# Autodesk Inventor assembly: om_AssemblyBody
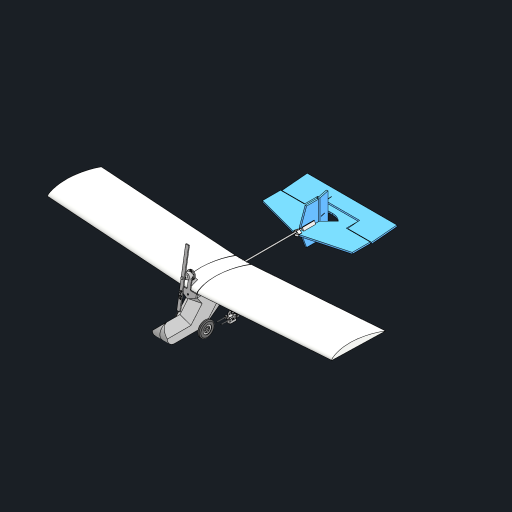
[picture p0: Inventor's stored thumbnail of the model, 512x512]
Saved by Autodesk Inventor 2023 (Build 270158000, 158)
## iProperties
Created: 2022-06-19
Part Number: om_AssemblyBody
Document SubType Name: Assembly
Designer: legot
Author: legot
## Documents named in this file (17)
- C:\Users\legot\OneDrive\ドキュメント\Inventor\HIKOSAPO\OM\om_HIKOROBO.iam
- C:\Users\legot\OneDrive\ドキュメント\Inventor\HIKOSAPO\OM\om_Body_L.ipt
- C:\Users\legot\OneDrive\ドキュメント\Inventor\HIKOSAPO\OM\om_Body_R.ipt
- C:\Users\legot\OneDrive\ドキュメント\Inventor\HIKOSAPO\OM\om_MotorMount.ipt
- C:\Users\legot\OneDrive\ドキュメント\Inventor\HIKOSAPO\public_parts\MainMotor.ipt
- C:\Users\legot\OneDrive\ドキュメント\Inventor\HIKOSAPO\public_parts\MainWing.ipt
- C:\Users\legot\OneDrive\ドキュメント\Inventor\HIKOSAPO\public_parts\Propeller.ipt
- C:\Users\legot\OneDrive\ドキュメント\Inventor\HIKOSAPO\public_parts\MainRod.ipt
- C:\Users\legot\OneDrive\ドキュメント\Inventor\HIKOSAPO\public_parts\HoriWing.ipt
- C:\Users\legot\OneDrive\ドキュメント\Inventor\HIKOSAPO\public_parts\HoriMove.ipt
- C:\Users\legot\OneDrive\ドキュメント\Inventor\HIKOSAPO\public_parts\VertMove.ipt
- C:\Users\legot\OneDrive\ドキュメント\Inventor\HIKOSAPO\public_parts\VertWing.ipt
- C:\Users\legot\OneDrive\ドキュメント\Inventor\HIKOSAPO\om_TailFrontHolder.ipt
- C:\Users\legot\OneDrive\ドキュメント\Inventor\HIKOSAPO\om_TailRod.ipt
- C:\Users\legot\OneDrive\ドキュメント\Inventor\HIKOSAPO\public_parts\Tire_Φ50.ipt
- C:\Users\legot\OneDrive\ドキュメント\Inventor\HIKOSAPO\public_parts\Wheel_Φ50.ipt
- C:\Users\legot\OneDrive\ドキュメント\Inventor\HIKOSAPO\DropMechanism\om_Drop.iam
## Components (18 placed, 16 different names)
1. om_Body_L:1 — フラッシュ:1, フラッシュ:3, フラッシュ:5, フラッシュ:6, メイト:1, メイト:2, フラッシュ:7, メイト:3
2. om_Body_R:1 — フラッシュ:2, フラッシュ:4, フラッシュ:6
3. om_MotorMount:1 — メイト:1, メイト:2, フラッシュ:7, 挿入:1, 挿入:2, 正接:1, フラッシュ:9, メイト:4, メイト:5
4. MainMotor:1 — 挿入:1, 挿入:2, 挿入:3
5. MainWing:1 — メイト:3, フラッシュ:8, 正接:1
6. Propeller:1 — 挿入:3
7. MainRod:1 — フラッシュ:9, メイト:4, メイト:5, フラッシュ:10, フラッシュ:11, フラッシュ:12, メイト:6, フラッシュ:13
8. HoriWing:1 — メイト:7, メイト:8, メイト:9, フラッシュ:14, メイト:10, メイト:15
9. HoriMove:1 — フラッシュ:14, メイト:10
10. VertMove:1 — メイト:14, フラッシュ:15
11. VertWing:1 — メイト:11, メイト:12, メイト:13, メイト:14, フラッシュ:15
12. om_TailFrontHolder:1 — フラッシュ:10, フラッシュ:12, メイト:15
13. om_TailRod:1 — フラッシュ:11, メイト:6, フラッシュ:13, メイト:7, メイト:8, メイト:9, メイト:11, メイト:12, メイト:13
14. Tire_Φ50:1 — メイト:16, メイト:17, フラッシュ:16
15. Tire_Φ50:2 — フラッシュ:17, フラッシュ:18, フラッシュ:19
16. Wheel_Φ50:1 — メイト:16, メイト:17, フラッシュ:16
17. Wheel_Φ50:2 — フラッシュ:17, フラッシュ:18, フラッシュ:19
18. om_Drop:1 [sub-assembly]
## Relationships (40: Flush 19, Mate 17, Insert 3, Tangent 1)
- フラッシュ:1 [Flush]: om_Body_L:1
- フラッシュ:2 [Flush]: om_Body_R:1
- フラッシュ:3 [Flush]: om_Body_L:1
- フラッシュ:4 [Flush]: om_Body_R:1
- フラッシュ:5 [Flush]: om_Body_L:1
- フラッシュ:6 [Flush]: om_Body_L:1 ↔ om_Body_R:1
- メイト:1 [Mate]: om_Body_L:1 ↔ om_MotorMount:1
- メイト:2 [Mate]: om_Body_L:1 ↔ om_MotorMount:1
- フラッシュ:7 [Flush]: om_Body_L:1 ↔ om_MotorMount:1
- 挿入:1 [Insert]: om_MotorMount:1 ↔ MainMotor:1
- 挿入:2 [Insert]: om_MotorMount:1 ↔ MainMotor:1
- メイト:3 [Mate]: om_Body_L:1 ↔ MainWing:1
- フラッシュ:8 [Flush]: MainWing:1
- 正接:1 [Tangent]: om_MotorMount:1 ↔ MainWing:1
- 挿入:3 [Insert]: MainMotor:1 ↔ Propeller:1
- フラッシュ:9 [Flush]: om_MotorMount:1 ↔ MainRod:1
- メイト:4 [Mate]: om_MotorMount:1 ↔ MainRod:1
- メイト:5 [Mate]: om_MotorMount:1 ↔ MainRod:1
- フラッシュ:10 [Flush]: MainRod:1 ↔ om_TailFrontHolder:1
- フラッシュ:11 [Flush]: MainRod:1 ↔ om_TailRod:1
- フラッシュ:12 [Flush]: MainRod:1 ↔ om_TailFrontHolder:1
- メイト:6 [Mate]: MainRod:1 ↔ om_TailRod:1
- フラッシュ:13 [Flush]: MainRod:1 ↔ om_TailRod:1
- メイト:7 [Mate]: HoriWing:1 ↔ om_TailRod:1
- メイト:8 [Mate]: HoriWing:1 ↔ om_TailRod:1
- メイト:9 [Mate]: HoriWing:1 ↔ om_TailRod:1
- フラッシュ:14 [Flush]: HoriWing:1 ↔ HoriMove:1
- メイト:10 [Mate]: HoriWing:1 ↔ HoriMove:1
- メイト:11 [Mate]: VertWing:1 ↔ om_TailRod:1
- メイト:12 [Mate]: VertWing:1 ↔ om_TailRod:1
- メイト:13 [Mate]: VertWing:1 ↔ om_TailRod:1
- メイト:14 [Mate]: VertMove:1 ↔ VertWing:1
- フラッシュ:15 [Flush]: VertMove:1 ↔ VertWing:1
- メイト:15 [Mate]: HoriWing:1 ↔ om_TailFrontHolder:1
- メイト:16 [Mate]: Tire_Φ50:1 ↔ Wheel_Φ50:1
- メイト:17 [Mate]: Tire_Φ50:1 ↔ Wheel_Φ50:1
- フラッシュ:16 [Flush]: Tire_Φ50:1 ↔ Wheel_Φ50:1
- フラッシュ:17 [Flush]: Tire_Φ50:2 ↔ Wheel_Φ50:2
- フラッシュ:18 [Flush]: Tire_Φ50:2 ↔ Wheel_Φ50:2
- フラッシュ:19 [Flush]: Tire_Φ50:2 ↔ Wheel_Φ50:2
